# Autodesk Inventor assembly: VeryBasicPitchingMachine
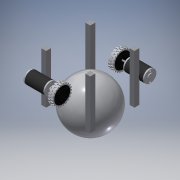
[picture p0: Inventor's stored thumbnail of the model, 180x180]
Saved by Autodesk Inventor 2016 SP1 (Build 200210100, 210)
## iProperties
Created: 2016-01-21
Part Number: VeryBasicPitchingMachine
Document SubType Name: Assembly
Designer: steele
Author: steele
## Documents named in this file (4)
- C:\snobotics\CAD-Development\robSteele\SnoBotics2016\2ndCutAtPitchingMachineRobot\VeryBasicPitchingMachine.iam
- C:\snobotics\CAD-Development\robSteele\SnoBotics2016\2ndCutAtPitchingMachineRobot\VeryBasicFrame.ipt
- C:\snobotics\CAD-Development\robSteele\SnoBotics2016\2ndCutAtPitchingMachineRobot\CimMotorAnd4inWheel.iam
- C:\snobotics\CAD-Development\robSteele\SnoBotics2016\DraftOfBoulder.ipt
## Components (4 placed, 3 different names)
1. VeryBasicFrame:1
2. CimMotorAnd4inWheel:1 [sub-assembly]
3. CimMotorAnd4inWheel:2 [sub-assembly]
4. DraftOfBoulder:1 — Mate:1, Mate:2
## Relationships (2: Mate 2)
- Mate:1: DraftOfBoulder:1
- Mate:2: DraftOfBoulder:1
